# Autodesk Inventor assembly: 201.001.01_ZB_Rahmen_GBG
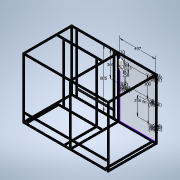
[picture p0: Inventor's stored thumbnail of the model, 180x180]
Saved by Autodesk Inventor 2022 (Build 260153000, 153)
## iProperties
Created: 2021-12-04
Part Number: 201.001.01_ZB_Rahmen_GBG
Document SubType Name: Assembly
Designer: Sebastian Seewald
Author: Sebastian Seewald
## Documents named in this file (33)
- C:\Users\kaebi\OneDrive - mci4me.at\03_MCI Master\4.Semester_SS2022\Masterarbeit\Software\CAD_TeachingFactory\201.001.01_ZB_Rahmen_GBG.iam
- C:\Users\kaebi\OneDrive - mci4me.at\03_MCI Master\4.Semester_SS2022\Masterarbeit\Software\CAD_TeachingFactory\101.001.01_Bodenplatte.ipt
- C:\Users\kaebi\OneDrive - mci4me.at\03_MCI Master\4.Semester_SS2022\Masterarbeit\Software\CAD_TeachingFactory\501.011.01_ITEM_20x20_N1_1160mm.ipt
- C:\Users\kaebi\OneDrive - mci4me.at\03_MCI Master\4.Semester_SS2022\Masterarbeit\Software\CAD_TeachingFactory\501.007.01_ITEM_20x20_N1_650mm.ipt
- 501.007.01_ITEM_20x20_N1_650mm.ipt
- C:\Users\kaebi\OneDrive - mci4me.at\03_MCI Master\4.Semester_SS2022\Masterarbeit\Software\CAD_TeachingFactory\501.001.01_ITEM_20x20_650mm.ipt
- 501.001.01_ITEM_20x20_650mm.ipt
- C:\Users\kaebi\OneDrive - mci4me.at\03_MCI Master\4.Semester_SS2022\Masterarbeit\Software\CAD_TeachingFactory\501.002.01_ITEM_20x20_630mm.ipt
- C:\Users\kaebi\OneDrive - mci4me.at\03_MCI Master\4.Semester_SS2022\Masterarbeit\Software\CAD_TeachingFactory\501.015.01_ITEM_20x20_438mm.ipt
- 501.015.01_ITEM_20x20_438mm.ipt
- C:\Users\kaebi\OneDrive - mci4me.at\03_MCI Master\4.Semester_SS2022\Masterarbeit\Software\CAD_TeachingFactory\501.013.01_ITEM_20x20_N2_850mm.ipt
- 501.013.01_ITEM_20x20_N2_850mm.ipt
- C:\Users\kaebi\OneDrive - mci4me.at\03_MCI Master\4.Semester_SS2022\Masterarbeit\Software\CAD_TeachingFactory\501.010.01_ITEM_20x20_N1_810mm.ipt
- 501.010.01_ITEM_20x20_N1_810mm.ipt
- C:\Users\kaebi\OneDrive - mci4me.at\03_MCI Master\4.Semester_SS2022\Masterarbeit\Software\CAD_TeachingFactory\501.014.01_ITEM_20x20_N2_1160mm.ipt
- C:\Users\kaebi\OneDrive - mci4me.at\03_MCI Master\4.Semester_SS2022\Masterarbeit\Software\CAD_TeachingFactory\501.012.01_ITEM_20x20_N2_650mm.ipt
- 501.012.01_ITEM_20x20_N2_650mm.ipt
- C:\Users\kaebi\OneDrive - mci4me.at\03_MCI Master\4.Semester_SS2022\Masterarbeit\Software\CAD_TeachingFactory\501.009.01_ITEM_20x20_N1_630mm.ipt
- C:\Users\kaebi\OneDrive - mci4me.at\03_MCI Master\4.Semester_SS2022\Masterarbeit\Software\CAD_TeachingFactory\501.016.01_ITEM_20x20_N2_630mm.ipt
- 501.013.01_ITEM_20x20_N2_630mm.ipt
- C:\Users\kaebi\OneDrive - mci4me.at\03_MCI Master\4.Semester_SS2022\Masterarbeit\Software\CAD_TeachingFactory\501.017.01_ITEM_20x20_N2_510mm.ipt
- 501.017.01_ITEM_20x20_N2_510mm.ipt
- C:\Users\kaebi\OneDrive - mci4me.at\03_MCI Master\4.Semester_SS2022\Masterarbeit\Software\CAD_TeachingFactory\501.018.01_Abdeckkappe_5_20x20.ipt
- C:\Users\kaebi\OneDrive - mci4me.at\03_MCI Master\4.Semester_SS2022\Masterarbeit\Software\CAD_TeachingFactory\501.019.01_ITEM_20x20_N2_505mm.ipt
- C:\Users\kaebi\OneDrive - mci4me.at\03_MCI Master\4.Semester_SS2022\Masterarbeit\Software\CAD_TeachingFactory\Acrly_Wand_1.ipt
- C:\Users\kaebi\OneDrive - mci4me.at\03_MCI Master\4.Semester_SS2022\Masterarbeit\Software\CAD_TeachingFactory\Acrly_Wand_3.ipt
- C:\Users\kaebi\OneDrive - mci4me.at\03_MCI Master\4.Semester_SS2022\Masterarbeit\Software\CAD_TeachingFactory\Acrly_Wand_4_1.ipt
- C:\Users\kaebi\OneDrive - mci4me.at\03_MCI Master\4.Semester_SS2022\Masterarbeit\Software\CAD_TeachingFactory\Acrly_Wand_6.ipt
- C:\Users\kaebi\OneDrive - mci4me.at\03_MCI Master\4.Semester_SS2022\Masterarbeit\Software\CAD_TeachingFactory\Acrly_Wand_7.ipt
- C:\Users\kaebi\OneDrive - mci4me.at\03_MCI Master\4.Semester_SS2022\Masterarbeit\Software\CAD_TeachingFactory\Acrly_Wand_8.ipt
- C:\Users\kaebi\OneDrive - mci4me.at\03_MCI Master\4.Semester_SS2022\Masterarbeit\Software\CAD_TeachingFactory\Acrly_Wand_9.ipt
- C:\Users\kaebi\OneDrive - mci4me.at\03_MCI Master\4.Semester_SS2022\Masterarbeit\Software\CAD_TeachingFactory\Tuere.iam
- C:\Users\kaebi\OneDrive - mci4me.at\03_MCI Master\4.Semester_SS2022\Masterarbeit\Software\CAD_TeachingFactory\101.003.01_Abdeckung_HMI_links.ipt
## Components (42 placed, 24 different names)
1. 101.001.01_Bodenplatte:1 — Fluchtend:1, Passend:1, Passend:2, Fluchtend:2, Passend:3, Passend:4, Fluchtend:3, Fluchtend:4, Passend:15, Fluchtend:11, Fluchtend:12, Passend:16, Fluchtend:13, Fluchtend:14, Passend:17, Fluchtend:15, Fluchtend:16, Passend:18, Fluchtend:17, Fluchtend:18
2. 501.011.01_ITEM_20x20_N1_1160mm:1 — Passend:3, Fluchtend:4, Passend:20, Passend:24, Passend:43, Passend:44, Passend:45, Fluchtend:47, Mate:58, Flush:53, Mate:60, Flush:54, Mate:74
3. 501.011.01_ITEM_20x20_N1_1160mm:2 — Fluchtend:1, Passend:1, Passend:5, Fluchtend:5, Passend:7, Fluchtend:7, Passend:10, Fluchtend:9, Passend:11, Fluchtend:10, Passend:22, Passend:23, Passend:37, Passend:38, Mate:64, Flush:56, Mate:66, Flush:57
4. 501.007.01_ITEM_20x20_N1_650mm:1 — Passend:2, Fluchtend:2, Passend:13, Passend:21, Mate:76
5. 501.007.01_ITEM_20x20_N1_650mm:2 — Passend:4, Fluchtend:3, Passend:6, Passend:19, Mate:53, Mate:55, Flush:51
6. 501.001.01_ITEM_20x20_650mm:1 — Passend:5, Fluchtend:5, Passend:6, Passend:9, Fluchtend:8, Fluchtend:19, Fluchtend:20
7. 501.001.01_ITEM_20x20_650mm:3 — Passend:7, Fluchtend:7, Mate:53
8. 501.002.01_ITEM_20x20_630mm:1 — Passend:9, Fluchtend:8, Passend:12, Fluchtend:33
9. 501.015.01_ITEM_20x20_438mm:1 — Passend:10, Fluchtend:9, Passend:13, Passend:14
10. 501.015.01_ITEM_20x20_438mm:2 — Passend:11, Fluchtend:10, Passend:12, Passend:14
11. 501.013.01_ITEM_20x20_N2_850mm:1 — Passend:17, Fluchtend:15, Fluchtend:16, Passend:19, Passend:20, Passend:26, Fluchtend:23, Fluchtend:24, Passend:27, Fluchtend:25, Fluchtend:26, Passend:41, Fluchtend:40, Fluchtend:41, Mate:72, Mate:73
12. 501.013.01_ITEM_20x20_N2_850mm:2 — Passend:16, Fluchtend:13, Fluchtend:14, Passend:21, Passend:40, Fluchtend:42, Fluchtend:43, Passend:48, Mate:61, Flush:60
13. 501.013.01_ITEM_20x20_N2_850mm:3 — Passend:15, Fluchtend:11, Fluchtend:12, Passend:25, Fluchtend:21, Fluchtend:22, Passend:28, Fluchtend:27, Fluchtend:28, Passend:39, Fluchtend:44, Fluchtend:45, Mate:65, Mate:75
14. 501.013.01_ITEM_20x20_N2_850mm:4 — Passend:18, Fluchtend:17, Fluchtend:18, Passend:22, Passend:35, Passend:42, Fluchtend:38, Fluchtend:39, Mate:54, Mate:67
15. 501.010.01_ITEM_20x20_N1_810mm:1 — Passend:24, Fluchtend:19, Fluchtend:29, Fluchtend:31, Mate:59
16. 501.010.01_ITEM_20x20_N1_810mm:2 — Passend:23, Fluchtend:20, Fluchtend:30, Passend:36, Fluchtend:36, Fluchtend:37
17. 501.014.01_ITEM_20x20_N2_1160mm:1 — Passend:26, Fluchtend:23, Fluchtend:24, Passend:29, Fluchtend:29, Mate:68, Flush:58, Mate:71
18. 501.014.01_ITEM_20x20_N2_1160mm:2 — Passend:25, Fluchtend:21, Fluchtend:22, Fluchtend:30
19. 501.012.01_ITEM_20x20_N2_650mm:1 — Passend:28, Fluchtend:27, Fluchtend:28, Passend:30, Fluchtend:32, Passend:51, Mate:70, Flush:59
20. 501.012.01_ITEM_20x20_N2_650mm:2 — Passend:27, Fluchtend:25, Fluchtend:26
21. 501.007.01_ITEM_20x20_N1_650mm:3 — Passend:29, Fluchtend:31, Mate:69
22. 501.009.01_ITEM_20x20_N1_630mm:1 — Passend:30, Fluchtend:32, Fluchtend:33, Passend:49, Passend:50, Fluchtend:49, Fluchtend:50
23. 501.013.01_ITEM_20x20_N2_630mm:1 — Passend:36, Fluchtend:36, Passend:37
24. 501.017.01_ITEM_20x20_N2_510mm:1 — Passend:35, Fluchtend:37, Passend:38
25. 501.018.01_Abdeckkappe_5_20x20:1 — Passend:39, Fluchtend:44, Fluchtend:45
26. 501.018.01_Abdeckkappe_5_20x20:2 — Passend:41, Fluchtend:40, Fluchtend:41
27. 501.018.01_Abdeckkappe_5_20x20:3 — Passend:40, Fluchtend:42, Fluchtend:43
28. 501.018.01_Abdeckkappe_5_20x20:4 — Passend:42, Fluchtend:38, Fluchtend:39
29. 501.019.01_ITEM_20x20_N2_505mm:1 — Passend:43, Passend:46, Passend:47, Fluchtend:46, Fluchtend:48
30. 501.010.01_ITEM_20x20_N1_810mm:3 — Passend:44, Passend:47, Fluchtend:47, Fluchtend:48
31. 501.010.01_ITEM_20x20_N1_810mm:4 — Passend:45, Passend:46, Fluchtend:46, Passend:48
32. 501.010.01_ITEM_20x20_N1_810mm:5 — Passend:50, Fluchtend:49, Passend:51, Passend:52
33. 501.010.01_ITEM_20x20_N1_810mm:6 — Passend:49, Fluchtend:50, Passend:52
34. Acrly_Wand_1:1 — Mate:54, Mate:55, Flush:51
35. Acrly_Wand_3:1 — Mate:58, Flush:53, Mate:59
36. Acrly_Wand_4_1:1 — Mate:60, Flush:54, Mate:61
37. Acrly_Wand_6:1 — Mate:64, Flush:56, Mate:65
38. Acrly_Wand_7:1 — Mate:66, Flush:57, Mate:67
39. Acrly_Wand_8:1 — Mate:68, Flush:58, Mate:69
40. Acrly_Wand_9:1 — Mate:70, Flush:59, Mate:71
41. Tuere:1 [sub-assembly] — Mate:72, Mate:73, Mate:74
42. 101.003.01_Abdeckung_HMI_links:1 — Mate:75, Mate:76, Flush:60
## Relationships (122: Mate 67, Flush 55)
- Fluchtend:1 [Flush]: 101.001.01_Bodenplatte:1 ↔ 501.011.01_ITEM_20x20_N1_1160mm:2
- Passend:1 [Mate]: 101.001.01_Bodenplatte:1 ↔ 501.011.01_ITEM_20x20_N1_1160mm:2
- Passend:2 [Mate]: 101.001.01_Bodenplatte:1 ↔ 501.007.01_ITEM_20x20_N1_650mm:1
- Fluchtend:2 [Flush]: 101.001.01_Bodenplatte:1 ↔ 501.007.01_ITEM_20x20_N1_650mm:1
- Passend:3 [Mate]: 101.001.01_Bodenplatte:1 ↔ 501.011.01_ITEM_20x20_N1_1160mm:1
- Passend:4 [Mate]: 101.001.01_Bodenplatte:1 ↔ 501.007.01_ITEM_20x20_N1_650mm:2
- Fluchtend:3 [Flush]: 101.001.01_Bodenplatte:1 ↔ 501.007.01_ITEM_20x20_N1_650mm:2
- Fluchtend:4 [Flush]: 101.001.01_Bodenplatte:1 ↔ 501.011.01_ITEM_20x20_N1_1160mm:1
- Passend:5 [Mate]: 501.011.01_ITEM_20x20_N1_1160mm:2 ↔ 501.001.01_ITEM_20x20_650mm:1
- Fluchtend:5 [Flush]: 501.011.01_ITEM_20x20_N1_1160mm:2 ↔ 501.001.01_ITEM_20x20_650mm:1
- Passend:6 [Mate] (510 mm): 501.007.01_ITEM_20x20_N1_650mm:2 ↔ 501.001.01_ITEM_20x20_650mm:1
- Passend:7 [Mate]: 501.011.01_ITEM_20x20_N1_1160mm:2 ↔ 501.001.01_ITEM_20x20_650mm:3
- Fluchtend:7 [Flush]: 501.011.01_ITEM_20x20_N1_1160mm:2 ↔ 501.001.01_ITEM_20x20_650mm:3
- Passend:9 [Mate]: 501.001.01_ITEM_20x20_650mm:1 ↔ 501.002.01_ITEM_20x20_630mm:1
- Fluchtend:8 [Flush]: 501.001.01_ITEM_20x20_650mm:1 ↔ 501.002.01_ITEM_20x20_630mm:1
- Passend:10 [Mate]: 501.011.01_ITEM_20x20_N1_1160mm:2 ↔ 501.015.01_ITEM_20x20_438mm:1
- Fluchtend:9 [Flush]: 501.011.01_ITEM_20x20_N1_1160mm:2 ↔ 501.015.01_ITEM_20x20_438mm:1
- Passend:11 [Mate]: 501.011.01_ITEM_20x20_N1_1160mm:2 ↔ 501.015.01_ITEM_20x20_438mm:2
- Fluchtend:10 [Flush]: 501.011.01_ITEM_20x20_N1_1160mm:2 ↔ 501.015.01_ITEM_20x20_438mm:2
- Passend:12 [Mate]: 501.002.01_ITEM_20x20_630mm:1 ↔ 501.015.01_ITEM_20x20_438mm:2
- Passend:13 [Mate] (10 mm): 501.007.01_ITEM_20x20_N1_650mm:1 ↔ 501.015.01_ITEM_20x20_438mm:1
- Passend:14 [Mate] (510 mm): 501.015.01_ITEM_20x20_438mm:1 ↔ 501.015.01_ITEM_20x20_438mm:2
- Passend:15 [Mate]: 101.001.01_Bodenplatte:1 ↔ 501.013.01_ITEM_20x20_N2_850mm:3
- Fluchtend:11 [Flush]: 101.001.01_Bodenplatte:1 ↔ 501.013.01_ITEM_20x20_N2_850mm:3
- Fluchtend:12 [Flush]: 101.001.01_Bodenplatte:1 ↔ 501.013.01_ITEM_20x20_N2_850mm:3
- Passend:16 [Mate]: 101.001.01_Bodenplatte:1 ↔ 501.013.01_ITEM_20x20_N2_850mm:2
- Fluchtend:13 [Flush]: 101.001.01_Bodenplatte:1 ↔ 501.013.01_ITEM_20x20_N2_850mm:2
- Fluchtend:14 [Flush]: 101.001.01_Bodenplatte:1 ↔ 501.013.01_ITEM_20x20_N2_850mm:2
- Passend:17 [Mate]: 101.001.01_Bodenplatte:1 ↔ 501.013.01_ITEM_20x20_N2_850mm:1
- Fluchtend:15 [Flush]: 101.001.01_Bodenplatte:1 ↔ 501.013.01_ITEM_20x20_N2_850mm:1
- Fluchtend:16 [Flush]: 101.001.01_Bodenplatte:1 ↔ 501.013.01_ITEM_20x20_N2_850mm:1
- Passend:18 [Mate]: 101.001.01_Bodenplatte:1 ↔ 501.013.01_ITEM_20x20_N2_850mm:4
- Fluchtend:17 [Flush]: 101.001.01_Bodenplatte:1 ↔ 501.013.01_ITEM_20x20_N2_850mm:4
- Fluchtend:18 [Flush]: 101.001.01_Bodenplatte:1 ↔ 501.013.01_ITEM_20x20_N2_850mm:4
- Passend:19 [Mate]: 501.007.01_ITEM_20x20_N1_650mm:2 ↔ 501.013.01_ITEM_20x20_N2_850mm:1
- Passend:20 [Mate]: 501.011.01_ITEM_20x20_N1_1160mm:1 ↔ 501.013.01_ITEM_20x20_N2_850mm:1
- Passend:21 [Mate]: 501.007.01_ITEM_20x20_N1_650mm:1 ↔ 501.013.01_ITEM_20x20_N2_850mm:2
- Passend:22 [Mate]: 501.011.01_ITEM_20x20_N1_1160mm:2 ↔ 501.013.01_ITEM_20x20_N2_850mm:4
- Passend:23 [Mate]: 501.011.01_ITEM_20x20_N1_1160mm:2 ↔ 501.010.01_ITEM_20x20_N1_810mm:2
- Passend:24 [Mate]: 501.011.01_ITEM_20x20_N1_1160mm:1 ↔ 501.010.01_ITEM_20x20_N1_810mm:1
- Fluchtend:19 [Flush]: 501.001.01_ITEM_20x20_650mm:1 ↔ 501.010.01_ITEM_20x20_N1_810mm:1
- Fluchtend:20 [Flush]: 501.001.01_ITEM_20x20_650mm:1 ↔ 501.010.01_ITEM_20x20_N1_810mm:2
- Passend:25 [Mate]: 501.013.01_ITEM_20x20_N2_850mm:3 ↔ 501.014.01_ITEM_20x20_N2_1160mm:2
- Fluchtend:21 [Flush]: 501.013.01_ITEM_20x20_N2_850mm:3 ↔ 501.014.01_ITEM_20x20_N2_1160mm:2
- Fluchtend:22 [Flush]: 501.013.01_ITEM_20x20_N2_850mm:3 ↔ 501.014.01_ITEM_20x20_N2_1160mm:2
- Passend:26 [Mate]: 501.013.01_ITEM_20x20_N2_850mm:1 ↔ 501.014.01_ITEM_20x20_N2_1160mm:1
- Fluchtend:23 [Flush]: 501.013.01_ITEM_20x20_N2_850mm:1 ↔ 501.014.01_ITEM_20x20_N2_1160mm:1
- Fluchtend:24 [Flush]: 501.013.01_ITEM_20x20_N2_850mm:1 ↔ 501.014.01_ITEM_20x20_N2_1160mm:1
- Passend:27 [Mate]: 501.013.01_ITEM_20x20_N2_850mm:1 ↔ 501.012.01_ITEM_20x20_N2_650mm:2
- Fluchtend:25 [Flush]: 501.013.01_ITEM_20x20_N2_850mm:1 ↔ 501.012.01_ITEM_20x20_N2_650mm:2
- Fluchtend:26 [Flush]: 501.013.01_ITEM_20x20_N2_850mm:1 ↔ 501.012.01_ITEM_20x20_N2_650mm:2
- Passend:28 [Mate]: 501.013.01_ITEM_20x20_N2_850mm:3 ↔ 501.012.01_ITEM_20x20_N2_650mm:1
- Fluchtend:27 [Flush]: 501.013.01_ITEM_20x20_N2_850mm:3 ↔ 501.012.01_ITEM_20x20_N2_650mm:1
- Fluchtend:28 [Flush]: 501.013.01_ITEM_20x20_N2_850mm:3 ↔ 501.012.01_ITEM_20x20_N2_650mm:1
- Passend:29 [Mate]: 501.014.01_ITEM_20x20_N2_1160mm:1 ↔ 501.007.01_ITEM_20x20_N1_650mm:3
- Fluchtend:29 [Flush]: 501.010.01_ITEM_20x20_N1_810mm:1 ↔ 501.014.01_ITEM_20x20_N2_1160mm:1
- Fluchtend:30 [Flush]: 501.010.01_ITEM_20x20_N1_810mm:2 ↔ 501.014.01_ITEM_20x20_N2_1160mm:2
- Fluchtend:31 [Flush]: 501.010.01_ITEM_20x20_N1_810mm:1 ↔ 501.007.01_ITEM_20x20_N1_650mm:3
- Passend:30 [Mate]: 501.012.01_ITEM_20x20_N2_650mm:1 ↔ 501.009.01_ITEM_20x20_N1_630mm:1
- Fluchtend:32 [Flush]: 501.012.01_ITEM_20x20_N2_650mm:1 ↔ 501.009.01_ITEM_20x20_N1_630mm:1
- Fluchtend:33 [Flush]: 501.002.01_ITEM_20x20_630mm:1 ↔ 501.009.01_ITEM_20x20_N1_630mm:1
- Passend:35 [Mate]: 501.013.01_ITEM_20x20_N2_850mm:4 ↔ 501.017.01_ITEM_20x20_N2_510mm:1
- Passend:36 [Mate]: 501.010.01_ITEM_20x20_N1_810mm:2 ↔ 501.013.01_ITEM_20x20_N2_630mm:1
- Fluchtend:36 [Flush]: 501.010.01_ITEM_20x20_N1_810mm:2 ↔ 501.013.01_ITEM_20x20_N2_630mm:1
- Fluchtend:37 [Flush]: 501.010.01_ITEM_20x20_N1_810mm:2 ↔ 501.017.01_ITEM_20x20_N2_510mm:1
- Passend:37 [Mate] (100 mm): 501.011.01_ITEM_20x20_N1_1160mm:2 ↔ 501.013.01_ITEM_20x20_N2_630mm:1
- Passend:38 [Mate] (100 mm): 501.011.01_ITEM_20x20_N1_1160mm:2 ↔ 501.017.01_ITEM_20x20_N2_510mm:1
- Passend:39 [Mate]: 501.013.01_ITEM_20x20_N2_850mm:3 ↔ 501.018.01_Abdeckkappe_5_20x20:1
- Passend:40 [Mate]: 501.013.01_ITEM_20x20_N2_850mm:2 ↔ 501.018.01_Abdeckkappe_5_20x20:3
- Passend:41 [Mate]: 501.013.01_ITEM_20x20_N2_850mm:1 ↔ 501.018.01_Abdeckkappe_5_20x20:2
- Passend:42 [Mate]: 501.013.01_ITEM_20x20_N2_850mm:4 ↔ 501.018.01_Abdeckkappe_5_20x20:4
- Fluchtend:38 [Flush]: 501.013.01_ITEM_20x20_N2_850mm:4 ↔ 501.018.01_Abdeckkappe_5_20x20:4
- Fluchtend:39 [Flush]: 501.013.01_ITEM_20x20_N2_850mm:4 ↔ 501.018.01_Abdeckkappe_5_20x20:4
- Fluchtend:40 [Flush]: 501.013.01_ITEM_20x20_N2_850mm:1 ↔ 501.018.01_Abdeckkappe_5_20x20:2
- Fluchtend:41 [Flush]: 501.013.01_ITEM_20x20_N2_850mm:1 ↔ 501.018.01_Abdeckkappe_5_20x20:2
- Fluchtend:42 [Flush]: 501.013.01_ITEM_20x20_N2_850mm:2 ↔ 501.018.01_Abdeckkappe_5_20x20:3
- Fluchtend:43 [Flush]: 501.013.01_ITEM_20x20_N2_850mm:2 ↔ 501.018.01_Abdeckkappe_5_20x20:3
- Fluchtend:44 [Flush]: 501.013.01_ITEM_20x20_N2_850mm:3 ↔ 501.018.01_Abdeckkappe_5_20x20:1
- Fluchtend:45 [Flush]: 501.013.01_ITEM_20x20_N2_850mm:3 ↔ 501.018.01_Abdeckkappe_5_20x20:1
- Passend:43 [Mate] (87.5 mm): 501.011.01_ITEM_20x20_N1_1160mm:1 ↔ 501.019.01_ITEM_20x20_N2_505mm:1
- Passend:44 [Mate]: 501.011.01_ITEM_20x20_N1_1160mm:1 ↔ 501.010.01_ITEM_20x20_N1_810mm:3
- Passend:45 [Mate]: 501.011.01_ITEM_20x20_N1_1160mm:1 ↔ 501.010.01_ITEM_20x20_N1_810mm:4
- Passend:46 [Mate]: 501.019.01_ITEM_20x20_N2_505mm:1 ↔ 501.010.01_ITEM_20x20_N1_810mm:4
- Passend:47 [Mate]: 501.019.01_ITEM_20x20_N2_505mm:1 ↔ 501.010.01_ITEM_20x20_N1_810mm:3
- Fluchtend:46 [Flush]: 501.019.01_ITEM_20x20_N2_505mm:1 ↔ 501.010.01_ITEM_20x20_N1_810mm:4
- Fluchtend:47 [Flush]: 501.011.01_ITEM_20x20_N1_1160mm:1 ↔ 501.010.01_ITEM_20x20_N1_810mm:3
- Fluchtend:48 [Flush]: 501.019.01_ITEM_20x20_N2_505mm:1 ↔ 501.010.01_ITEM_20x20_N1_810mm:3
- Passend:48 [Mate] (47.5 mm): 501.013.01_ITEM_20x20_N2_850mm:2 ↔ 501.010.01_ITEM_20x20_N1_810mm:4
- Passend:49 [Mate]: 501.009.01_ITEM_20x20_N1_630mm:1 ↔ 501.010.01_ITEM_20x20_N1_810mm:6
- Passend:50 [Mate]: 501.009.01_ITEM_20x20_N1_630mm:1 ↔ 501.010.01_ITEM_20x20_N1_810mm:5
- Fluchtend:49 [Flush]: 501.009.01_ITEM_20x20_N1_630mm:1 ↔ 501.010.01_ITEM_20x20_N1_810mm:5
- Fluchtend:50 [Flush]: 501.009.01_ITEM_20x20_N1_630mm:1 ↔ 501.010.01_ITEM_20x20_N1_810mm:6
- Passend:51 [Mate] (80 mm): 501.012.01_ITEM_20x20_N2_650mm:1 ↔ 501.010.01_ITEM_20x20_N1_810mm:5
- Passend:52 [Mate] (440 mm): 501.010.01_ITEM_20x20_N1_810mm:5 ↔ 501.010.01_ITEM_20x20_N1_810mm:6
- Mate:53 (30 mm): 501.007.01_ITEM_20x20_N1_650mm:2 ↔ 501.001.01_ITEM_20x20_650mm:3
- Mate:54: 501.013.01_ITEM_20x20_N2_850mm:4 ↔ Acrly_Wand_1:1
- Mate:55: 501.007.01_ITEM_20x20_N1_650mm:2 ↔ Acrly_Wand_1:1
- Flush:51 (7.5 mm): 501.007.01_ITEM_20x20_N1_650mm:2 ↔ Acrly_Wand_1:1
- Mate:58: 501.011.01_ITEM_20x20_N1_1160mm:1 ↔ Acrly_Wand_3:1
- Flush:53 (7.5 mm): 501.011.01_ITEM_20x20_N1_1160mm:1 ↔ Acrly_Wand_3:1
- Mate:59 (-6.35 mm): 501.010.01_ITEM_20x20_N1_810mm:1 ↔ Acrly_Wand_3:1
- Mate:60: 501.011.01_ITEM_20x20_N1_1160mm:1 ↔ Acrly_Wand_4_1:1
- Flush:54 (7.5 mm): 501.011.01_ITEM_20x20_N1_1160mm:1 ↔ Acrly_Wand_4_1:1
- Mate:61 (-6.35 mm): 501.013.01_ITEM_20x20_N2_850mm:2 ↔ Acrly_Wand_4_1:1
- Mate:64: 501.011.01_ITEM_20x20_N1_1160mm:2 ↔ Acrly_Wand_6:1
- Flush:56 (7.5 mm): 501.011.01_ITEM_20x20_N1_1160mm:2 ↔ Acrly_Wand_6:1
- Mate:65: 501.013.01_ITEM_20x20_N2_850mm:3 ↔ Acrly_Wand_6:1
- Mate:66: 501.011.01_ITEM_20x20_N1_1160mm:2 ↔ Acrly_Wand_7:1
- Flush:57 (7.5 mm): 501.011.01_ITEM_20x20_N1_1160mm:2 ↔ Acrly_Wand_7:1
- Mate:67: 501.013.01_ITEM_20x20_N2_850mm:4 ↔ Acrly_Wand_7:1
- Mate:68: 501.014.01_ITEM_20x20_N2_1160mm:1 ↔ Acrly_Wand_8:1
- Flush:58 (7.5 mm): 501.014.01_ITEM_20x20_N2_1160mm:1 ↔ Acrly_Wand_8:1
- Mate:69: 501.007.01_ITEM_20x20_N1_650mm:3 ↔ Acrly_Wand_8:1
- Mate:70: 501.012.01_ITEM_20x20_N2_650mm:1 ↔ Acrly_Wand_9:1
- Flush:59 (7.5 mm): 501.012.01_ITEM_20x20_N2_650mm:1 ↔ Acrly_Wand_9:1
- Mate:71: 501.014.01_ITEM_20x20_N2_1160mm:1 ↔ Acrly_Wand_9:1
- Mate:72: 501.013.01_ITEM_20x20_N2_850mm:1 ↔ Tuere:1
- Mate:73 (-20 mm): 501.013.01_ITEM_20x20_N2_850mm:1 ↔ Tuere:1
- Mate:74: 501.011.01_ITEM_20x20_N1_1160mm:1 ↔ Tuere:1
- Mate:75: 501.013.01_ITEM_20x20_N2_850mm:3 ↔ 101.003.01_Abdeckung_HMI_links:1
- Mate:76: 501.007.01_ITEM_20x20_N1_650mm:1 ↔ 101.003.01_Abdeckung_HMI_links:1
- Flush:60 (7.5 mm): 501.013.01_ITEM_20x20_N2_850mm:2 ↔ 101.003.01_Abdeckung_HMI_links:1
